# Autodesk Inventor assembly: 組合1
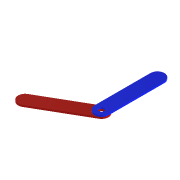
[picture p0: Inventor's stored thumbnail of the model, 180x180]
Saved by Autodesk Inventor 2022 (Build 260153000, 153)
## iProperties
Created: 2023-04-19
Part Number: 組合1
Document SubType Name: Assembly
Designer: JOU
Author: JOU
## Documents named in this file (2)
- C:\Users\JOU\Desktop\git\Special-project\ppt用\組合1.iam
- C:\Users\JOU\Desktop\git\Special-project\ppt用\零件1.ipt
## Components (2 placed, 1 different names)
1. 零件1:1 — 插入:1, 角度:1
2. 零件1:2 — 插入:1, 角度:1
## Relationships (2: Insert 1, Angle 1)
- 插入:1 [Insert]: 零件1:1 ↔ 零件1:2
- 角度:1 [Angle] (420 deg): 零件1:1 ↔ 零件1:2
